# Autodesk Inventor assembly: Car_Assembly
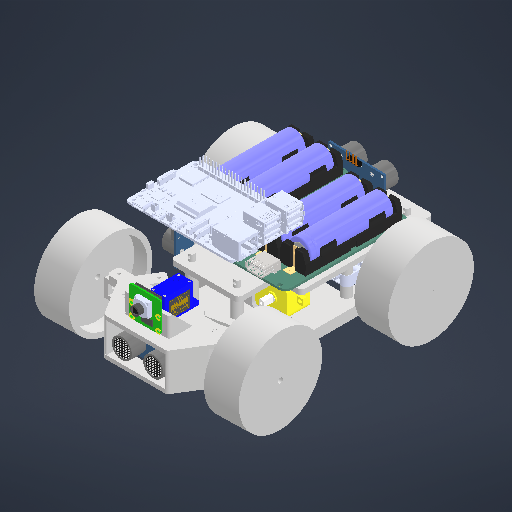
[picture p0: Inventor's stored thumbnail of the model, 512x512]
Saved by Autodesk Inventor 2025 (Build 290162010, 162A)
## iProperties
Created: 2024-05-24
Part Number: Car_Assembly
Document SubType Name: Assembly
Designer: Garfieldcmix
Author: Garfieldcmix
## Documents named in this file (26)
- C:\Users\chaya\Desktop\WRO-2024-CAD\Inventor\Car_Assembly.iam
- C:\Users\chaya\Desktop\WRO-2024-CAD\Inventor\SG90 - Micro Servo 9g - Tower Pro\SG90 - Micro Servo 9g - Tower Pro.iam
- C:\Users\chaya\Desktop\WRO-2024-CAD\Inventor\Front_Bridge.ipt
- C:\Users\chaya\Desktop\WRO-2024-CAD\Inventor\SG90 - Micro Servo 9g - Tower Pro\SG90 - Micro Servo 9g - Tower Pro.2.ipt
- C:\Users\chaya\Desktop\WRO-2024-CAD\Inventor\Front_Wheel_Anchor.ipt
- C:\Users\chaya\Desktop\WRO-2024-CAD\Inventor\Front_Wheel_Anchor_MIR.ipt
- C:\Users\chaya\Desktop\WRO-2024-CAD\Inventor\Wheel.ipt
- C:\Users\chaya\Desktop\WRO-2024-CAD\Inventor\Wheel_MIR.ipt
- C:\Users\chaya\Desktop\WRO-2024-CAD\Inventor\Pi camera module3\Pi camera module3.ipt
- C:\Users\chaya\Desktop\WRO-2024-CAD\Inventor\4519 DkStone Technic Axle 3\4519 DkStone Technic Axle 3.ipt
- C:\Users\chaya\Desktop\WRO-2024-CAD\Inventor\Lego Beam Fram 5x7 (64179)\Lego Beam Fram 5x7 (64179).ipt
- C:\Users\chaya\Desktop\WRO-2024-CAD\Inventor\TT Motor\TT Motor.ipt
- C:\Users\chaya\Desktop\WRO-2024-CAD\Inventor\Lower_Chassis.ipt
- C:\Users\chaya\Desktop\WRO-2024-CAD\Inventor\Motor_Lego_Axle_Connector.ipt
- C:\Users\chaya\Desktop\WRO-2024-CAD\Inventor\Wheel_Lego_Axle_Connector.ipt
- C:\Users\chaya\Desktop\WRO-2024-CAD\Inventor\Front_Bridge_2.ipt
- C:\Users\chaya\Desktop\WRO-2024-CAD\Inventor\Servo_Steering_Linkage.ipt
- C:\Users\chaya\Desktop\WRO-2024-CAD\Inventor\hc-sr04\hc-sr04.iam
- C:\Users\chaya\Desktop\WRO-2024-CAD\Inventor\Lego_Frame_Holder.ipt
- C:\Users\chaya\Desktop\WRO-2024-CAD\Inventor\Lego_Frame_Holder_Extra.ipt
- C:\Users\chaya\Desktop\WRO-2024-CAD\Inventor\Lego_Frame_Holder_Extra_2.ipt
- C:\Users\chaya\Desktop\WRO-2024-CAD\Inventor\1.5_base.ipt
- C:\Users\chaya\Desktop\WRO-2024-CAD\Inventor\18650 2-WAY v5\18650 2-WAY v5.iam
- C:\Users\chaya\Desktop\WRO-2024-CAD\Inventor\MAKER-DRIVE\MAKER-DRIVE.iam
- C:\Users\chaya\Desktop\WRO-2024-CAD\Inventor\MPU_6050\MPU_6050.iam
- C:\Users\chaya\Desktop\WRO-2024-CAD\Inventor\RASPBERRY_PI_5\RASPBERRY_PI_5.iam
## Components (42 placed, 32 different names)
1. 1.5_base:1 — Mate:125, Mate:126, Mate:127, Mate:128
2. 18650 2-WAY v5:1 [sub-assembly]
3. 18650 2-WAY v5:2 [sub-assembly]
4. MAKER-DRIVE:1 [sub-assembly]
5. hc-sr04:2 [sub-assembly]
6. hc-sr04:3 [sub-assembly]
7. MPU_6050:1 [sub-assembly]
8. RASPBERRY_PI_5:1 [sub-assembly]
9. Pi camera module3:1 — Mate:73, Mate:72, Mate:74
10. hc-sr04:1 [sub-assembly] — Mate:92, Mate:93, Mate:94
11. SG90_Servo [sub-assembly] — Mate:1, Mate:16, Mate:2, Mate:17, Mate:69
12. Left_Servo_Steering_Linkage — Mate:83, Mate:84, Mate:85, Mate:86
13. Right_Servo_Steering_Linkage — Mate:87, Mate:88, Mate:89, Mate:90
14. Front_Bridge:1 — Mate:38, Mate:39, Mate:40, Mate:41, Mate:42, Mate:66, Mate:67, Mate:68, Mate:75, Mate:76, Mate:79, Mate:80, Angle:1, Mate:92, Mate:93, Mate:94
15. Front_Bridge_2:1 — Mate:66, Mate:67, Mate:68, Mate:69, Mate:73, Mate:72, Mate:74, Mate:1, Mate:16
16. Left_Front_Wheel_Anchor — Mate:75, Mate:76, Mate:77, Mate:78, Mate:83, Mate:85, Angle:1
17. Left_Front_Wheel — Mate:77, Mate:78
18. Right_Front_Wheel_Anchor — Mate:79, Mate:80, Mate:81, Mate:82, Mate:88, Mate:89
19. Right_Front_Wheel — Mate:81, Mate:82
20. Servo_Arm — Mate:2, Mate:17, Mate:84, Mate:86, Mate:87, Mate:90
21. Lower_Chassis:1 — Mate:38, Mate:39, Mate:40, Mate:41, Mate:42, Mate:43, Mate:44, Mate:45, Mate:46, Mate:47, Mate:48, Mate:57, Mate:91, Mate:96, Mate:97, Mate:98, Mate:100, Mate:101, Mate:103, Mate:104, Mate:106, Mate:107, Mate:109, Mate:110, Mate:112, Mate:113, Mate:115, Mate:116, Mate:118, Mate:119, Mate:120, Mate:121, Mate:122, Mate:123, Mate:124
22. Left_Lego_Beam_Frame — Mate:37, Mate:43, Mate:44, Mate:45, Mate:50, Mate:55, Mate:60, Mate:102, Mate:105, Mate:108, Mate:117
23. Lego_Driving_Shaft_Axle — Mate:50, Mate:53, Mate:54
24. TT Motor:1 — Mate:51, Mate:52, Mate:57, Mate:91
25. Motor_Lego_Axle_Connector — Mate:51, Mate:52, Mate:53, Mate:54, Mate:55
26. Right_Lego_Beam_Frame — Mate:46, Mate:47, Mate:48, Mate:49, Mate:63, Mate:95, Mate:99, Mate:111, Mate:114
27. Left_Lego_Wheel_Axle — Mate:37, Mate:58, Mate:59
28. Left_Wheel_Lego_Axle_Connector — Mate:58, Mate:59, Mate:60, Mate:64, Flush:3
29. Left_Back_Wheel — Mate:64, Flush:3
30. Right_Lego_Wheel_Axle — Mate:49, Mate:61, Mate:62
31. Right_Wheel_Lego_Axle_Connector — Mate:61, Mate:62, Mate:63, Mate:65, Flush:4
32. Right_Back_Wheel — Mate:65, Flush:4
33. Lego_Frame_Holder:1 — Mate:95, Mate:96, Mate:97
34. Lego_Frame_Holder:2 — Mate:98, Mate:99, Mate:100
35. Lego_Frame_Holder:3 — Mate:101, Mate:102, Mate:103
36. Lego_Frame_Holder:4 — Mate:104, Mate:105, Mate:106
37. Lego_Frame_Holder:5 — Mate:107, Mate:108, Mate:109
38. Lego_Frame_Holder:6 — Mate:110, Mate:111, Mate:112
39. Lego_Frame_Holder_Extra:1 — Mate:113, Mate:114, Mate:115
40. Lego_Frame_Holder_Extra:2 — Mate:116, Mate:117, Mate:118, Mate:125, Mate:128
41. Lego_Frame_Holder_Extra_2:1 — Mate:119, Mate:120, Mate:121
42. Lego_Frame_Holder_Extra_2:2 — Mate:122, Mate:123, Mate:124, Mate:126, Mate:127
## Relationships (96: Mate 93, Flush 2, Angle 1)
- Mate:1: SG90_Servo ↔ Front_Bridge_2:1
- Mate:16: SG90_Servo ↔ Front_Bridge_2:1
- Mate:2: SG90_Servo ↔ Servo_Arm
- Mate:17: SG90_Servo ↔ Servo_Arm
- Mate:37: Left_Lego_Beam_Frame ↔ Left_Lego_Wheel_Axle
- Mate:38: Front_Bridge:1 ↔ Lower_Chassis:1
- Mate:39: Front_Bridge:1 ↔ Lower_Chassis:1
- Mate:40: Front_Bridge:1 ↔ Lower_Chassis:1
- Mate:41: Front_Bridge:1 ↔ Lower_Chassis:1
- Mate:42: Front_Bridge:1 ↔ Lower_Chassis:1
- Mate:43: Lower_Chassis:1 ↔ Left_Lego_Beam_Frame
- Mate:44: Lower_Chassis:1 ↔ Left_Lego_Beam_Frame
- Mate:45: Lower_Chassis:1 ↔ Left_Lego_Beam_Frame
- Mate:46: Lower_Chassis:1 ↔ Right_Lego_Beam_Frame
- Mate:47: Lower_Chassis:1 ↔ Right_Lego_Beam_Frame
- Mate:48: Lower_Chassis:1 ↔ Right_Lego_Beam_Frame
- Mate:49: Right_Lego_Beam_Frame ↔ Right_Lego_Wheel_Axle
- Mate:50: Left_Lego_Beam_Frame ↔ Lego_Driving_Shaft_Axle
- Mate:51: TT Motor:1 ↔ Motor_Lego_Axle_Connector
- Mate:52: TT Motor:1 ↔ Motor_Lego_Axle_Connector
- Mate:53: Lego_Driving_Shaft_Axle ↔ Motor_Lego_Axle_Connector
- Mate:54: Lego_Driving_Shaft_Axle ↔ Motor_Lego_Axle_Connector
- Mate:55: Left_Lego_Beam_Frame ↔ Motor_Lego_Axle_Connector
- Mate:57: Lower_Chassis:1 ↔ TT Motor:1
- Mate:58: Left_Lego_Wheel_Axle ↔ Left_Wheel_Lego_Axle_Connector
- Mate:59: Left_Lego_Wheel_Axle ↔ Left_Wheel_Lego_Axle_Connector
- Mate:60: Left_Lego_Beam_Frame ↔ Left_Wheel_Lego_Axle_Connector
- Mate:61: Right_Lego_Wheel_Axle ↔ Right_Wheel_Lego_Axle_Connector
- Mate:62: Right_Lego_Wheel_Axle ↔ Right_Wheel_Lego_Axle_Connector
- Mate:63: Right_Lego_Beam_Frame ↔ Right_Wheel_Lego_Axle_Connector
- Mate:64: Left_Wheel_Lego_Axle_Connector ↔ Left_Back_Wheel
- Flush:3: Left_Wheel_Lego_Axle_Connector ↔ Left_Back_Wheel
- Mate:65: Right_Wheel_Lego_Axle_Connector ↔ Right_Back_Wheel
- Flush:4: Right_Wheel_Lego_Axle_Connector ↔ Right_Back_Wheel
- Mate:66: Front_Bridge:1 ↔ Front_Bridge_2:1
- Mate:67: Front_Bridge:1 ↔ Front_Bridge_2:1
- Mate:68: Front_Bridge:1 ↔ Front_Bridge_2:1
- Mate:69: SG90_Servo ↔ Front_Bridge_2:1
- Mate:73: Pi camera module3:1 ↔ Front_Bridge_2:1
- Mate:72: Pi camera module3:1 ↔ Front_Bridge_2:1
- Mate:74: Pi camera module3:1 ↔ Front_Bridge_2:1
- Mate:75: Front_Bridge:1 ↔ Left_Front_Wheel_Anchor
- Mate:76: Front_Bridge:1 ↔ Left_Front_Wheel_Anchor
- Mate:77: Left_Front_Wheel_Anchor ↔ Left_Front_Wheel
- Mate:78: Left_Front_Wheel_Anchor ↔ Left_Front_Wheel
- Mate:79: Front_Bridge:1 ↔ Right_Front_Wheel_Anchor
- Mate:80: Front_Bridge:1 ↔ Right_Front_Wheel_Anchor
- Mate:81: Right_Front_Wheel_Anchor ↔ Right_Front_Wheel
- Mate:82: Right_Front_Wheel_Anchor ↔ Right_Front_Wheel
- Mate:83: Left_Servo_Steering_Linkage ↔ Left_Front_Wheel_Anchor
- Mate:84: Left_Servo_Steering_Linkage ↔ Servo_Arm
- Mate:85: Left_Servo_Steering_Linkage ↔ Left_Front_Wheel_Anchor
- Angle:1 (180 deg): Front_Bridge:1 ↔ Left_Front_Wheel_Anchor
- Mate:86: Left_Servo_Steering_Linkage ↔ Servo_Arm
- Mate:87: Right_Servo_Steering_Linkage ↔ Servo_Arm
- Mate:88: Right_Servo_Steering_Linkage ↔ Right_Front_Wheel_Anchor
- Mate:89: Right_Servo_Steering_Linkage ↔ Right_Front_Wheel_Anchor
- Mate:90: Right_Servo_Steering_Linkage ↔ Servo_Arm
- Mate:91: Lower_Chassis:1 ↔ TT Motor:1
- Mate:92: hc-sr04:1 ↔ Front_Bridge:1
- Mate:93: hc-sr04:1 ↔ Front_Bridge:1
- Mate:94: hc-sr04:1 ↔ Front_Bridge:1
- Mate:95: Right_Lego_Beam_Frame ↔ Lego_Frame_Holder:1
- Mate:96: Lower_Chassis:1 ↔ Lego_Frame_Holder:1
- Mate:97: Lower_Chassis:1 ↔ Lego_Frame_Holder:1
- Mate:98: Lower_Chassis:1 ↔ Lego_Frame_Holder:2
- Mate:99: Right_Lego_Beam_Frame ↔ Lego_Frame_Holder:2
- Mate:100: Lower_Chassis:1 ↔ Lego_Frame_Holder:2
- Mate:101: Lower_Chassis:1 ↔ Lego_Frame_Holder:3
- Mate:102: Left_Lego_Beam_Frame ↔ Lego_Frame_Holder:3
- Mate:103: Lower_Chassis:1 ↔ Lego_Frame_Holder:3
- Mate:104: Lower_Chassis:1 ↔ Lego_Frame_Holder:4
- Mate:105: Left_Lego_Beam_Frame ↔ Lego_Frame_Holder:4
- Mate:106: Lower_Chassis:1 ↔ Lego_Frame_Holder:4
- Mate:107: Lower_Chassis:1 ↔ Lego_Frame_Holder:5
- Mate:108: Left_Lego_Beam_Frame ↔ Lego_Frame_Holder:5
- Mate:109: Lower_Chassis:1 ↔ Lego_Frame_Holder:5
- Mate:110: Lower_Chassis:1 ↔ Lego_Frame_Holder:6
- Mate:111: Right_Lego_Beam_Frame ↔ Lego_Frame_Holder:6
- Mate:112: Lower_Chassis:1 ↔ Lego_Frame_Holder:6
- Mate:113: Lower_Chassis:1 ↔ Lego_Frame_Holder_Extra:1
- Mate:114: Right_Lego_Beam_Frame ↔ Lego_Frame_Holder_Extra:1
- Mate:115: Lower_Chassis:1 ↔ Lego_Frame_Holder_Extra:1
- Mate:116: Lower_Chassis:1 ↔ Lego_Frame_Holder_Extra:2
- Mate:117: Left_Lego_Beam_Frame ↔ Lego_Frame_Holder_Extra:2
- Mate:118: Lower_Chassis:1 ↔ Lego_Frame_Holder_Extra:2
- Mate:119: Lower_Chassis:1 ↔ Lego_Frame_Holder_Extra_2:1
- Mate:120: Lower_Chassis:1 ↔ Lego_Frame_Holder_Extra_2:1
- Mate:121: Lower_Chassis:1 ↔ Lego_Frame_Holder_Extra_2:1
- Mate:122: Lower_Chassis:1 ↔ Lego_Frame_Holder_Extra_2:2
- Mate:123: Lower_Chassis:1 ↔ Lego_Frame_Holder_Extra_2:2
- Mate:124: Lower_Chassis:1 ↔ Lego_Frame_Holder_Extra_2:2
- Mate:125: 1.5_base:1 ↔ Lego_Frame_Holder_Extra:2
- Mate:126: 1.5_base:1 ↔ Lego_Frame_Holder_Extra_2:2
- Mate:127: 1.5_base:1 ↔ Lego_Frame_Holder_Extra_2:2
- Mate:128: 1.5_base:1 ↔ Lego_Frame_Holder_Extra:2
